# Autodesk Inventor assembly: base
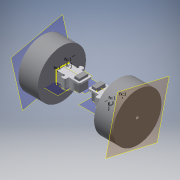
[picture p0: Inventor's stored thumbnail of the model, 180x180]
Saved by Autodesk Inventor 2018 (Build 220112000, 112)
## iProperties
Created: 2017-09-29
Part Number: base
Document SubType Name: Assembly
Designer: fabre
d0: 0,000 mm
d1: 0,000 mm
base_L: 50,000 mm
wheel_shaft_percentage: 0,315 ul
pico_dist: 15,000 mm
laser: 0,400 mm
thick: 4,990 mm
d11: 0,000 mm
d12: -74,000 mm
d13: 0,000 mm
base_fix_holes_dist: 7,000 mm
extra_wood: 3,327 mm
pen_d: 20,000 mm
fente_l: 15,437 mm
nb_fentes: 2,000 ul
male_l: 16,237 mm
batt_hole_l: 35,000 mm
finger_l: 17,000 mm
chepeau_L: 74,990 mm
vis_moteur_d: 2,600 mm
cale_d: 5,000 mm
charniere_epaisseur_axe: 2,600 mm
charniere_trou_d: 2,500 mm
charniere_distance_trou: 8,250 mm
charniere_ecart: 17,200 mm
charniere_L: 24,100 mm
inclinaison: 10,00 deg
tete_hole_margin: 0,100 mm
chanfrein: 1,000 mm
charniere_edge2hole: 7,800 mm
etage_height: 10,000 mm
motor_height: 10,000 mm
motor_width: 12,000 mm
extrud1: 22,400 mm
d3: 0,00 deg
d4: 3,000 mm
d5: 9,000 mm
d6: 0,00 deg
d7: 17,000 mm
extrud3: 6,400 mm
d9: 0,00 deg
Author: fabre
## Documents named in this file (3)
- C:\Users\rfabre\Desktop\cubi\mechanics\pendulum\base.iam
- C:\Users\rfabre\Desktop\cubi\mechanics\pendulum\motor_block.iam
- C:\Users\rfabre\Desktop\cubi\mechanics\pendulum\motor.ipt
## Components (2 placed, 1 different names)
1. motor_block:1 [sub-assembly] — Flush:1, Flush:2, Mate:1, Mate:2, Mate:3
2. motor_block:2 [sub-assembly] — Flush:1, Mate:1, Mate:2
## Relationships (5: Mate 3, Flush 2)
- Flush:1: motor_block:1 ↔ motor_block:2
- Flush:2: motor_block:1
- Mate:1: motor_block:1 ↔ motor_block:2
- Mate:2 (-74 mm): motor_block:1 ↔ motor_block:2
- Mate:3: motor_block:1
## Named parameters: base_L = 70 mm, wheel_shaft_percentage = 0.315, pico_dist = 15 mm, laser = 0.4 mm, thick = 4.99 mm, base_fix_holes_dist = 7 mm, extra_wood = 3.32667 mm, pen_d = 20 mm, fente_l = 4.59 mm, nb_fentes = 2, fente_L = 15.43667 mm, male_l = 5.39 mm, male_L = 16.23667 mm, batt_hole_l = 15 mm, batt_hole_L = 35 mm, finger_l = 10 mm, finger_L = 17 mm, chepeau_L = 74.99 mm, vis_moteur_d = 2.6 mm, cale_d = 5 mm, charniere_epaisseur_axe = 2.6 mm, charniere_trou_d = 2.5 mm, charniere_distance_trou = 8.25 mm, charniere_ecart = 17.2 mm, charniere_L = 24.1 mm, tete_hole_margin = 0.1 mm, inclinaison = 10 deg, chanfrein = 1 mm, charniere_edge2hole = 7.8 mm, base_l = 50 mm, etage_height = 10 mm, motor_height = 10 mm, motor_width = 12 mm, extrud1 = 22.4 mm, extrud3 = 6.4 mm
